# Autodesk Inventor assembly: NDV-3400 Branch 4 01
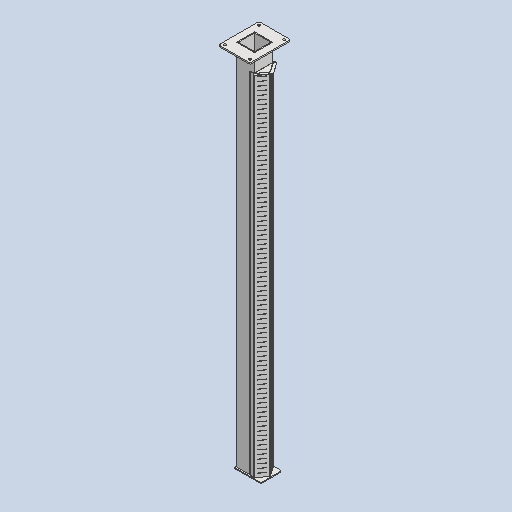
[picture p0: Inventor's stored thumbnail of the model, 512x512]
Saved by Autodesk Inventor 2026.2 (Build 302298000, 298)
## iProperties
Created: 2026-10-05
Part Number: NDV-3400 Branch 4 01
Document SubType Name: Assembly
Designer: admin
Stock Number: Луч 4
Author: admin
## Documents named in this file (6)
- C:\Users\admin\Documents\Inventor\NDV-DistribSystem\DRS_D1200\NDV-3400 Branch 4 01.iam
- C:\Users\admin\Documents\Inventor\NDV-DistribSystem\DRS_D1200\NDV-3401 Branch tube 04.ipt
- C:\Users\admin\Documents\Inventor\NDV-DistribSystem\DRS_D1200\NDV-3001 Branch flange 01.ipt
- C:\Users\admin\Documents\Inventor\NDV-DistribSystem\DRS_D1200\NDV-3402 Branch roof 04.ipt
- C:\Users\admin\Documents\Inventor\NDV-DistribSystem\DRS_D1200\NDV-3002 Branch cap 01.ipt
- C:\Users\admin\Documents\Inventor\NDV-DistribSystem\DRS_D1200\NDV-3003 Branch roof cap 01.ipt
## Components (5 placed, 5 different names)
1. NDV-3401 Branch tube 04:1 — Flush:1, Mate:1, Mate:2, Flush:2, Mate:3, Mate:4, Mate:5, Flush:3, Flush:4, Mate:7, Flush:5
2. NDV-3001 Branch flange 01:1 — Flush:1, Mate:1, Mate:2
3. NDV-3402 Branch roof 04:1 — Flush:2, Mate:3, Mate:4, Mate:6
4. NDV-3002 Branch cap 01:1 — Mate:5, Flush:3, Flush:4
5. NDV-3003 Branch roof cap 01:1 — Mate:6, Mate:7, Flush:5
## Relationships (12: Mate 7, Flush 5)
- Flush:1: NDV-3401 Branch tube 04:1 ↔ NDV-3001 Branch flange 01:1
- Mate:1 (0.1 mm): NDV-3401 Branch tube 04:1 ↔ NDV-3001 Branch flange 01:1
- Mate:2 (0.1 mm): NDV-3401 Branch tube 04:1 ↔ NDV-3001 Branch flange 01:1
- Flush:2: NDV-3401 Branch tube 04:1 ↔ NDV-3402 Branch roof 04:1
- Mate:3 (0.1576 mm): NDV-3401 Branch tube 04:1 ↔ NDV-3402 Branch roof 04:1
- Mate:4 (-9.5 mm): NDV-3401 Branch tube 04:1 ↔ NDV-3402 Branch roof 04:1
- Mate:5: NDV-3401 Branch tube 04:1 ↔ NDV-3002 Branch cap 01:1
- Flush:3 (-3 mm): NDV-3401 Branch tube 04:1 ↔ NDV-3002 Branch cap 01:1
- Flush:4 (-2 mm): NDV-3401 Branch tube 04:1 ↔ NDV-3002 Branch cap 01:1
- Mate:6: NDV-3402 Branch roof 04:1 ↔ NDV-3003 Branch roof cap 01:1
- Mate:7: NDV-3401 Branch tube 04:1 ↔ NDV-3003 Branch roof cap 01:1
- Flush:5: NDV-3401 Branch tube 04:1 ↔ NDV-3003 Branch roof cap 01:1
